# Autodesk Inventor assembly: assembly_connector
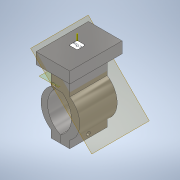
[picture p0: Inventor's stored thumbnail of the model, 180x180]
Saved by Autodesk Inventor 2021 (Build 250183000, 183)
## iProperties
Created: 2021-05-17
Part Number: assembly_connector
Document SubType Name: Assembly
Designer: chick
Author: chick
## Documents named in this file (9)
- C:\Users\chick\OneDrive - Flinders\Chi Ki Siu Work\CAD work\initial_design_connector\assembly_connector_left_part_and_hinge.0002.iam
- C:\Users\chick\OneDrive - Flinders\Chi Ki Siu Work\CAD work\initial_design_connector\connector_base.0004.ipt
- C:\Users\chick\OneDrive - Flinders\Chi Ki Siu Work\CAD work\initial_design_connector\hinge.0005.ipt
- C:\Users\chick\OneDrive - Flinders\Chi Ki Siu Work\CAD work\initial_design_connector\assembly_connector_left_part_and_hinge.0002\AIP\FEA\dm8jgjkn4.fins
- C:\Users\chick\OneDrive - Flinders\Chi Ki Siu Work\CAD work\initial_design_connector\assembly_connector_left_part_and_hinge.0002\AIP\FEA\dm8jgjkn4.fsat
- C:\Users\chick\OneDrive - Flinders\Chi Ki Siu Work\CAD work\initial_design_connector\assembly_connector_left_part_and_hinge.0002\AIP\FEA\dm8jgjkn4.ftes
- C:\Users\chick\OneDrive - Flinders\Chi Ki Siu Work\CAD work\initial_design_connector\assembly_connector_left_part_and_hinge.0002\AIP\FEA\dm8jgjkn4.fwiz
- C:\Users\chick\OneDrive - Flinders\Chi Ki Siu Work\CAD work\initial_design_connector\assembly_connector_left_part_and_hinge.0002\AIP\FEA\dm8jgjko0.fmsh
- C:\Users\chick\OneDrive - Flinders\Chi Ki Siu Work\CAD work\initial_design_connector\assembly_connector_left_part_and_hinge.0002\AIP\FEA\dm8jgjko1.fres
## Components (2 placed, 2 different names)
1. connector_base.0004:1 — Mate:1, Mate:2
2. hinge.0005:1 — Mate:1, Mate:2
## Relationships (2: Mate 2)
- Mate:1: connector_base.0004:1 ↔ hinge.0005:1
- Mate:2: connector_base.0004:1 ↔ hinge.0005:1
## Named parameters: sa_0 = 98000, sa_1 = 5000
note: some values were not read from the file. Shown as the stored number, unit unknown: "sa_0", "sa_1".
